# Autodesk Inventor assembly: ADSK-MH-10046
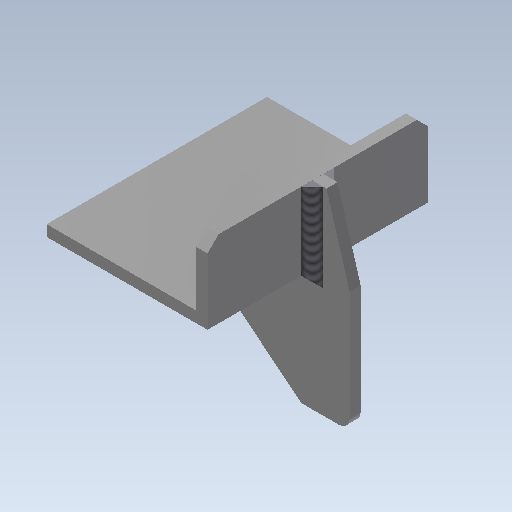
[picture p0: Inventor's stored thumbnail of the model, 512x512]
Saved by Autodesk Inventor 2020.2 (Build 242310000, 310)
## iProperties
Created: 2008-03-27
Part Number: ADSK-MH-10046
Document SubType Name: Weldment
Designer: R.O'mahony
Weld Material: Welded Aluminum-6061
Description: Support Bracket Weldment
Engineer: Demir Ali
Checked By: Demir Ali
Company: Autodesk Ltd
Author: R.O'mahony
Keywords: Roller Conveyor
Revision Number: A
## Documents named in this file (3)
- C:\Users\peter\source\repos\InventorDA-FLC\Dataset\Discharge Conveyor\ADSK-MH-10046.iam
- C:\Users\peter\source\repos\InventorDA-FLC\Dataset\Discharge Conveyor\ADSK-MH-10039.ipt
- C:\Users\peter\source\repos\InventorDA-FLC\Dataset\Discharge Conveyor\ADSK-MH-10040.ipt
## Components (2 placed, 2 different names)
1. ADSK-MH-10039:1 — Flush:1, Mate:1
2. ADSK-MH-10040:1 — Flush:1, Mate:1
## Relationships (2: Flush 1, Mate 1)
- Flush:1: ADSK-MH-10039:1 ↔ ADSK-MH-10040:1
- Mate:1: ADSK-MH-10039:1 ↔ ADSK-MH-10040:1
